# Autodesk Inventor assembly: assembly_support
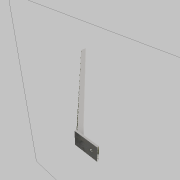
[picture p0: Inventor's stored thumbnail of the model, 180x180]
Saved by Autodesk Inventor 2021 (Build 250183000, 183)
## iProperties
Created: 2021-05-11
Part Number: assembly_support
Document SubType Name: Assembly
Designer: Watchdog
Author: Watchdog
## Documents named in this file (3)
- C:\Users\Watchdog\OneDrive - Flinders\Advn Mech Design Shared\6_Development\2_Design\inventor\support\assembly_support.iam
- C:\Users\Watchdog\OneDrive - Flinders\Advn Mech Design Shared\6_Development\2_Design\inventor\support\support_weldPlate.ipt
- C:\Users\Watchdog\OneDrive - Flinders\Advn Mech Design Shared\6_Development\2_Design\inventor\support\bar_square_500mm_25sides_hollow_cut45deg.ipt
## Components (2 placed, 2 different names)
1. support_weldPlate:2 — Mate:2, Mate:3, Flush:1, Mate:4, Angle:1, Mate:5
2. bar_square_500mm_25sides_hollow_cut45deg:1 — Mate:3, Angle:1, Mate:5
## Relationships (6: Mate 4, Flush 1, Angle 1)
- Mate:2: support_weldPlate:2
- Mate:3: support_weldPlate:2 ↔ bar_square_500mm_25sides_hollow_cut45deg:1
- Flush:1: support_weldPlate:2
- Mate:4: support_weldPlate:2
- Angle:1 (180 deg): support_weldPlate:2 ↔ bar_square_500mm_25sides_hollow_cut45deg:1
- Mate:5: support_weldPlate:2 ↔ bar_square_500mm_25sides_hollow_cut45deg:1
